# Autodesk Inventor assembly: Привод
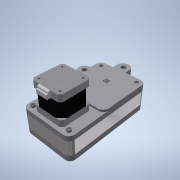
[picture p0: Inventor's stored thumbnail of the model, 180x180]
Saved by Autodesk Inventor 2021 (Build 250183000, 183)
## iProperties
Created: 2020-12-07
Part Number: Привод
Document SubType Name: Assembly
Designer: User
Mass: 935.322 g
Surface Area: 1230.71 cm^2
Volume: 304.227 cm^3
Density: 3.07442 g/cm^3
Author: User
## Documents named in this file (12)
- F:\Vise\Модели\Тиски\Привод.iam
- F:\Vise\Модели\Тиски\Тиски\Мастер проектирования\Цилиндрическое зубчатое зацепление5.iam
- F:\Vise\Модели\Тиски\Привод\Мастер проектирования\Цилиндрическое зубчатое зацепление2.iam
- F:\Vise\Модели\Тиски\Шаговый двигатель.ipt
- C:\Users\User\Documents\Inventor\Content Center Files\R2020\ru-RU\DIN 913\DIN 913 - M3 x 6.ipt
- F:\Vise\Модели\Тиски\Привод\Мастер проектирования\Подшипник1.iam
- F:\Vise\Модели\Тиски\Привод\Мастер проектирования\Подшипник2.iam
- F:\Vise\Модели\Тиски\Пластина 1.ipt
- F:\Vise\Модели\Тиски\Пластина 2.ipt
- F:\Vise\Модели\Тиски\Стойка.ipt
- F:\Vise\Модели\Тиски\Привод\Мастер проектирования\Болтовое соединение4.iam
- C:\Users\User\Documents\Inventor\Content Center Files\R2021\ru-RU\AS 1427(05)\AS 1427 - M6 x 35(5) II.ipt
## Components (17 placed, 9 different names)
1. Цилиндрическое зубчатое зацепление:1 [sub-assembly] — С поворотом:1, Совмещение:1, Совмещение:2, Совмещение:3, Совмещение:4, Совмещение:7, Жесткий:3, Заподлицо:1, С поворотом:5
2. Цилиндрическое зубчатое зацепление:2 [sub-assembly] — С поворотом:1, Совмещение:8, Жесткий:1, Жесткий:2, С поворотом:2, С поворотом:3, С поворотом:4, Заподлицо:2
3. Шаговый двигатель:1 — Совмещение:13, С поворотом:2
4. DIN 913 M3 x 6:1 — Жесткий:1
5. DIN 913 M3 x 6:2 — Жесткий:2
6. Подшипник:1 [sub-assembly] — Жесткий:3
7. Подшипник:2 [sub-assembly] — С поворотом:5
8. Подшипник:3 [sub-assembly] — С поворотом:3
9. Подшипник:4 [sub-assembly] — С поворотом:4
10. Пластина 1:1 — Заподлицо:1, Совмещение:30, Совмещение:31
11. Пластина 2:1 — Заподлицо:2, Заподлицо:3, Заподлицо:4, Совмещение:14, Совмещение:15, Совмещение:16, Совмещение:17, Совмещение:18, Совмещение:20, Совмещение:22, Совмещение:24, С поворотом:6, С поворотом:7, С поворотом:8, С поворотом:9
12. Болтовое соединение:3 [sub-assembly] — Совмещение:30, Совмещение:31
13. AS 1427 H - метрическая M6 x 35:1 — С поворотом:9
14. AS 1427 H - метрическая M6 x 35:2 — С поворотом:6
15. AS 1427 H - метрическая M6 x 35:3 — С поворотом:7
16. AS 1427 H - метрическая M6 x 35:4 — С поворотом:8
17. Стойка:1 — Заподлицо:3, Заподлицо:4
## Relationships (42: Mate 26, RevoluteJoint 9, Flush 4, WeldJoint 3)
- С поворотом:1 [RevoluteJoint]: Цилиндрическое зубчатое зацепление:1 ↔ Цилиндрическое зубчатое зацепление:2
- Совмещение:1 [Mate]: Цилиндрическое зубчатое зацепление:1
- Совмещение:2 [Mate]: Цилиндрическое зубчатое зацепление:1
- Совмещение:3 [Mate]: Цилиндрическое зубчатое зацепление:1
- Совмещение:4 [Mate]: Цилиндрическое зубчатое зацепление:1
- Совмещение:5 [Mate]
- Совмещение:6 [Mate]
- Совмещение:7 [Mate]: Цилиндрическое зубчатое зацепление:1
- Совмещение:8 [Mate]: Цилиндрическое зубчатое зацепление:2
- Совмещение:9 [Mate]
- Совмещение:10 [Mate]
- Совмещение:11 [Mate]
- Совмещение:13 [Mate]: Шаговый двигатель:1
- Жесткий:1 [WeldJoint] (0.2 mm): Цилиндрическое зубчатое зацепление:2 ↔ DIN 913 M3 x 6:1
- Жесткий:2 [WeldJoint]: Цилиндрическое зубчатое зацепление:2 ↔ DIN 913 M3 x 6:2
- Жесткий:3 [WeldJoint]: Цилиндрическое зубчатое зацепление:1 ↔ Подшипник:1
- С поворотом:2 [RevoluteJoint] (-8 mm): Цилиндрическое зубчатое зацепление:2 ↔ Шаговый двигатель:1
- С поворотом:3 [RevoluteJoint]: Цилиндрическое зубчатое зацепление:2 ↔ Подшипник:3
- С поворотом:4 [RevoluteJoint]: Цилиндрическое зубчатое зацепление:2 ↔ Подшипник:4
- Заподлицо:1 [Flush]: Цилиндрическое зубчатое зацепление:1 ↔ Пластина 1:1
- Заподлицо:2 [Flush]: Цилиндрическое зубчатое зацепление:2 ↔ Пластина 2:1
- Заподлицо:3 [Flush]: Пластина 2:1 ↔ Стойка:1
- Заподлицо:4 [Flush]: Пластина 2:1 ↔ Стойка:1
- Совмещение:14 [Mate]: Пластина 2:1
- Совмещение:15 [Mate]: Пластина 2:1
- Совмещение:16 [Mate]: Пластина 2:1
- Совмещение:17 [Mate]: Пластина 2:1
- Совмещение:18 [Mate]: Пластина 2:1
- Совмещение:19 [Mate]
- Совмещение:20 [Mate]: Пластина 2:1
- Совмещение:21 [Mate]
- Совмещение:22 [Mate]: Пластина 2:1
- Совмещение:23 [Mate]
- Совмещение:24 [Mate]: Пластина 2:1
- Совмещение:25 [Mate]
- С поворотом:5 [RevoluteJoint]: Цилиндрическое зубчатое зацепление:1 ↔ Подшипник:2
- Совмещение:30 [Mate]: Пластина 1:1 ↔ Болтовое соединение:3
- Совмещение:31 [Mate]: Пластина 1:1 ↔ Болтовое соединение:3
- С поворотом:6 [RevoluteJoint]: Пластина 2:1 ↔ AS 1427 H - метрическая M6 x 35:2
- С поворотом:7 [RevoluteJoint]: Пластина 2:1 ↔ AS 1427 H - метрическая M6 x 35:3
- С поворотом:8 [RevoluteJoint]: Пластина 2:1 ↔ AS 1427 H - метрическая M6 x 35:4
- С поворотом:9 [RevoluteJoint]: Пластина 2:1 ↔ AS 1427 H - метрическая M6 x 35:1
